# Autodesk Inventor assembly: Index_Finger_assembly_1
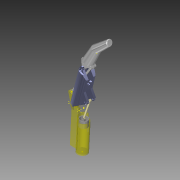
[picture p0: Inventor's stored thumbnail of the model, 180x180]
Saved by Autodesk Inventor 2015 (Build 190159000, 159)
## iProperties
Created: 2016-07-06
Part Number: Index_Finger_assembly_1
Document SubType Name: Assembly
Designer: Neelotpal Nag
Mass: 10.1916 g
Surface Area: 106.91 cm^2
Volume: 10.1916 cm^3
Density: 1 g/cm^3
Author: Neelotpal Nag
## Documents named in this file (7)
- D:\DISA 2016\Fingers 1\Index_Finger_assembly_1.iam
- D:\DISA 2016\Fingers 1\Base_Cylinder_1.ipt
- D:\DISA 2016\Fingers 1\Cylinder_1.ipt
- D:\DISA 2016\Fingers 1\Finger_Lower_main_1.ipt
- D:\DISA 2016\Fingers 1\Finger_Upper_main_1.ipt
- D:\DISA 2016\Fingers 1\Restrain_Pin_1.ipt
- D:\DISA 2016\Fingers 1\Shaft_Piston.ipt
## Components (6 placed, 6 different names)
1. Base_Cylinder_1:1 — Mate:4, Mate:5, Mate:16, Mate:17, Mate:19, Angle:1
2. Cylinder_1:1 — Mate:13, Mate:14, Mate:19, Angle:1
3. Finger_Lower_main_1:1 — Mate:4, Mate:5, Mate:7, Mate:8, Mate:15
4. Finger_Upper_main_1:1 — Mate:7, Mate:8, Mate:18
5. Shaft_Piston:1 — Mate:13, Mate:14, Mate:15
6. Restrain_Pin_1:1 — Mate:16, Mate:17, Mate:18
## Relationships (12: Mate 11, Angle 1)
- Mate:4: Base_Cylinder_1:1 ↔ Finger_Lower_main_1:1
- Mate:5: Base_Cylinder_1:1 ↔ Finger_Lower_main_1:1
- Mate:7 (0.5 mm): Finger_Lower_main_1:1 ↔ Finger_Upper_main_1:1
- Mate:8: Finger_Lower_main_1:1 ↔ Finger_Upper_main_1:1
- Mate:13: Cylinder_1:1 ↔ Shaft_Piston:1
- Mate:14: Cylinder_1:1 ↔ Shaft_Piston:1
- Mate:15: Finger_Lower_main_1:1 ↔ Shaft_Piston:1
- Mate:16: Base_Cylinder_1:1 ↔ Restrain_Pin_1:1
- Mate:17 (0.05 mm): Base_Cylinder_1:1 ↔ Restrain_Pin_1:1
- Mate:18: Finger_Upper_main_1:1 ↔ Restrain_Pin_1:1
- Mate:19: Base_Cylinder_1:1 ↔ Cylinder_1:1
- Angle:1 (0 deg): Base_Cylinder_1:1 ↔ Cylinder_1:1
